# Autodesk Inventor assembly: esp_holder_assemble
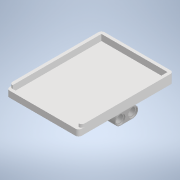
[picture p0: Inventor's stored thumbnail of the model, 180x180]
Saved by Autodesk Inventor 2021 (Build 250183000, 183)
## iProperties
Created: 2024-05-29
Part Number: esp_holder_assemble
Document SubType Name: Assembly
Designer: 23adrdam
Author: 23adrdam
## Documents named in this file (3)
- C:\Users\23adrdam\Desktop\driverbot\driverbot-adrian\models\esp_holder_assemble.iam
- C:\Users\23adrdam\Downloads\Imported Components\BEAM 2_\BEAM 2_.ipt
- C:\Users\23adrdam\Desktop\driverbot\driverbot-adrian\models\esp_shield_holder.ipt
## Components (3 placed, 2 different names)
1. BEAM 2_:1 — Mate:2, Mate:3
2. esp_shield_holder:1 — Mate:1, Mate:2
3. BEAM 2_:2 — Mate:1, Mate:3
## Relationships (3: Mate 3)
- Mate:1: esp_shield_holder:1 ↔ BEAM 2_:2
- Mate:2: BEAM 2_:1 ↔ esp_shield_holder:1
- Mate:3: BEAM 2_:1 ↔ BEAM 2_:2
